# Autodesk Inventor assembly: trussstructure
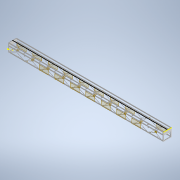
[picture p0: Inventor's stored thumbnail of the model, 180x180]
Saved by Autodesk Inventor 2020 (Build 240168000, 168)
## iProperties
Created: 2020-07-04
Part Number: trussstructure
Document SubType Name: Assembly
Designer: Ashiqrahman
Mass: 1909.65 g
Surface Area: 18631.2 cm^2
Volume: 1909.65 cm^3
Density: 1 g/cm^3
Author: Ashiqrahman
## Documents named in this file (12)
- D:\projects\Intelligent Picking\trussstructure.iam
- D:\projects\Intelligent Picking\LINK 2 tri truss without horizontal members.ipt
- C:\Users\Public\Documents\Autodesk\Inventor 2020\truss frame slanting.ipt
- C:\Users\Public\Documents\Autodesk\Inventor 2020\truss frame slanting down.ipt
- C:\Users\Public\Documents\Autodesk\Inventor 2020\truss final piece.ipt
- C:\Users\Public\Documents\Autodesk\Inventor 2020\horizontal bottom trusses.ipt
- C:\Users\Public\Documents\Autodesk\Inventor 2020\horizontal truss top.ipt
- D:\projects\Intelligent Picking\trussstructure\AIP\FEA\dajo7qeu8.fins
- D:\projects\Intelligent Picking\trussstructure\AIP\FEA\dajo7qeu8.fsat
- D:\projects\Intelligent Picking\trussstructure\AIP\FEA\dajo7qeu8.ftes
- D:\projects\Intelligent Picking\trussstructure\AIP\FEA\dajo7qeu8.fwiz
- D:\projects\Intelligent Picking\trussstructure\AIP\FEA\dajo7qeww.fmsh
## Components (60 placed, 6 different names)
1. LINK 2 tri truss without horizontal members:1 — Rotational:1, Mate:1, Mate:2, Mate:3, Flush:3, Flush:4, Mate:4, Mate:5, Flush:5, Mate:6, Mate:7, Mate:8, Mate:9, Flush:6, Mate:10, Mate:11, Flush:7, Mate:12, Mate:13, Flush:8, Mate:14, Mate:15, Flush:9, Mate:16, Mate:17, Flush:10, Mate:18, Mate:19, Flush:11, Mate:36, Mate:37, Flush:21, Mate:38, Mate:39, Flush:22, Mate:40, Flush:23, Mate:41, Mate:42, Flush:24, Mate:43, Mate:44, Mate:45, Mate:46, Mate:47, Flush:25, Mate:48, Mate:49, Flush:26, Mate:50, Mate:51, Flush:27, Mate:52, Mate:53, Flush:28, Mate:54, Mate:56, Mate:74, Flush:40, Mate:75, Flush:41, Mate:76, Mate:78, Flush:43, Flush:44, Flush:45, Mate:79, Mate:80, Flush:46, Mate:82, Mate:83, Flush:47, Mate:84, Mate:85, Flush:48, Mate:86, Mate:87, Mate:88, Flush:49, Mate:89, Mate:90, Flush:50, Mate:91, Mate:92, Flush:51, Mate:93, Mate:94, Flush:52, Mate:95, Mate:96, Flush:53, Mate:97, Mate:98, Flush:54, Flush:55, Flush:56, Mate:99, Mate:100, Flush:57, Mate:101, Mate:102, Flush:58, Mate:103, Mate:104, Flush:59, Mate:105, Mate:106, Flush:60, Mate:107, Mate:108, Flush:61, Mate:109, Mate:110, Flush:62, Mate:111, Mate:112, Flush:63, Mate:113, Mate:114, Flush:64, Mate:115, Mate:116, Flush:65
2. truss frame slanting:1 — Flush:2, Rotational:1, Mate:1, Mate:20
3. truss frame slanting down:1 — Flush:2, Mate:20, Mate:21
4. truss frame slanting:2 — Mate:2, Mate:3, Flush:3, Mate:21, Mate:22, Flush:12
5. truss frame slanting:3 — Mate:18, Mate:19, Flush:11, Mate:35, Mate:77, Flush:42
6. truss frame slanting:4 — Flush:4, Mate:4, Mate:5, Mate:23, Flush:13
7. truss frame slanting:5 — Mate:16, Mate:17, Flush:10, Mate:32, Mate:33, Flush:19
8. truss frame slanting:6 — Mate:12, Mate:13, Flush:8, Mate:28, Mate:29, Flush:17
9. truss frame slanting:7 — Mate:14, Mate:15, Flush:9, Mate:30, Mate:31, Flush:18
10. truss frame slanting:8 — Flush:5, Mate:6, Mate:7, Mate:24
11. truss frame slanting:9 — Mate:10, Mate:11, Flush:7, Mate:27, Flush:16
12. truss frame slanting:10 — Mate:8, Mate:9, Flush:6, Mate:25, Flush:14, Mate:26, Flush:15
13. truss frame slanting down:2 — Mate:24, Mate:25, Flush:14
14. truss frame slanting down:3 — Mate:23, Flush:13
15. truss frame slanting down:4 — Mate:22, Flush:12
16. truss frame slanting down:5 — Mate:26, Flush:15
17. truss frame slanting down:6 — Mate:27, Flush:16, Mate:28
18. truss frame slanting down:7 — Mate:29, Flush:17, Mate:30
19. truss frame slanting down:8 — Mate:31, Flush:18, Mate:32
20. truss frame slanting down:9 — Mate:33, Flush:19, Mate:35
21. truss frame slanting down:11 — Mate:44, Mate:45, Mate:46, Mate:64, Mate:65, Flush:34
22. truss frame slanting down:12 — Mate:40, Flush:23, Mate:41, Mate:60, Mate:61, Flush:32
23. truss frame slanting down:13 — Mate:36, Mate:37, Flush:21, Mate:55, Flush:29, Mate:58
24. truss frame slanting down:14 — Mate:38, Mate:39, Flush:22, Mate:57, Flush:30, Mate:59, Flush:31
25. truss frame slanting down:15 — Mate:42, Flush:24, Mate:43, Mate:62, Mate:63, Flush:33
26. truss frame slanting down:16 — Mate:47, Flush:25, Mate:48, Flush:35, Mate:66, Mate:67, Flush:36
27. truss frame slanting down:17 — Mate:49, Flush:26, Mate:50, Mate:68, Mate:69, Flush:37
28. truss frame slanting down:18 — Mate:51, Flush:27, Mate:52, Mate:70, Mate:71, Flush:38
29. truss frame slanting down:19 — Mate:53, Flush:28, Mate:54, Mate:72, Mate:73, Flush:39
30. truss frame slanting:11 — Mate:63, Flush:33, Mate:64
31. truss frame slanting:12 — Mate:65, Flush:34, Flush:35, Mate:66
32. truss frame slanting:13 — Mate:59, Flush:31, Mate:60
33. truss frame slanting:14 — Mate:55, Flush:29, Mate:56
34. truss frame slanting:15 — Mate:67, Flush:36, Mate:68
35. truss frame slanting:16 — Mate:61, Flush:32, Mate:62
36. truss frame slanting:17 — Mate:57, Flush:30, Mate:58
37. truss frame slanting:18 — Mate:69, Flush:37, Mate:70
38. truss frame slanting:19 — Mate:71, Flush:38, Mate:72
39. truss frame slanting:20 — Mate:73, Flush:39, Mate:74
40. truss final piece:1 — Flush:40, Mate:75, Flush:41, Mate:76
41. truss final piece:2 — Mate:77, Flush:42, Mate:78
42. horizontal bottom trusses:1 — Flush:43, Flush:44, Flush:45, Mate:79, Mate:80, Flush:46
43. horizontal bottom trusses:2 — Mate:91, Mate:92, Flush:51
44. horizontal bottom trusses:3 — Mate:84, Mate:85, Flush:48
45. horizontal bottom trusses:4 — Mate:89, Mate:90, Flush:50
46. horizontal bottom trusses:5 — Mate:86, Mate:87, Mate:88, Flush:49
47. horizontal bottom trusses:6 — Mate:95, Mate:96, Flush:53
48. horizontal bottom trusses:7 — Mate:93, Mate:94, Flush:52
49. horizontal bottom trusses:8 — Mate:82, Mate:83, Flush:47
50. horizontal bottom trusses:9 — Mate:97, Mate:98, Flush:54
51. horizontal truss top:1 — Flush:55, Flush:56
52. horizontal truss top:2 — Mate:99, Mate:100, Flush:57
53. horizontal truss top:3 — Mate:101, Mate:102, Flush:58
54. horizontal truss top:4 — Mate:103, Mate:104, Flush:59
55. horizontal truss top:5 — Mate:105, Mate:106, Flush:60
56. horizontal truss top:6 — Mate:107, Mate:108, Flush:61
57. horizontal truss top:7 — Mate:109, Mate:110, Flush:62
58. horizontal truss top:8 — Mate:111, Mate:112, Flush:63
59. horizontal truss top:9 — Mate:113, Mate:114, Flush:64
60. horizontal truss top:10 — Mate:115, Mate:116, Flush:65
## Relationships (178: Mate 114, Flush 63, RevoluteJoint 1)
- Flush:2: truss frame slanting:1 ↔ truss frame slanting down:1
- Rotational:1 [RevoluteJoint]: LINK 2 tri truss without horizontal members:1 ↔ truss frame slanting:1
- Mate:1: LINK 2 tri truss without horizontal members:1 ↔ truss frame slanting:1
- Mate:2: LINK 2 tri truss without horizontal members:1 ↔ truss frame slanting:2
- Mate:3: LINK 2 tri truss without horizontal members:1 ↔ truss frame slanting:2
- Flush:3 (-3 mm): LINK 2 tri truss without horizontal members:1 ↔ truss frame slanting:2
- Flush:4 (-3 mm): LINK 2 tri truss without horizontal members:1 ↔ truss frame slanting:4
- Mate:4: LINK 2 tri truss without horizontal members:1 ↔ truss frame slanting:4
- Mate:5: LINK 2 tri truss without horizontal members:1 ↔ truss frame slanting:4
- Flush:5 (-3 mm): LINK 2 tri truss without horizontal members:1 ↔ truss frame slanting:8
- Mate:6: LINK 2 tri truss without horizontal members:1 ↔ truss frame slanting:8
- Mate:7: LINK 2 tri truss without horizontal members:1 ↔ truss frame slanting:8
- Mate:8: LINK 2 tri truss without horizontal members:1 ↔ truss frame slanting:10
- Mate:9: LINK 2 tri truss without horizontal members:1 ↔ truss frame slanting:10
- Flush:6 (-3 mm): LINK 2 tri truss without horizontal members:1 ↔ truss frame slanting:10
- Mate:10: LINK 2 tri truss without horizontal members:1 ↔ truss frame slanting:9
- Mate:11: LINK 2 tri truss without horizontal members:1 ↔ truss frame slanting:9
- Flush:7 (-3 mm): LINK 2 tri truss without horizontal members:1 ↔ truss frame slanting:9
- Mate:12: LINK 2 tri truss without horizontal members:1 ↔ truss frame slanting:6
- Mate:13: LINK 2 tri truss without horizontal members:1 ↔ truss frame slanting:6
- Flush:8 (3 mm): LINK 2 tri truss without horizontal members:1 ↔ truss frame slanting:6
- Mate:14: LINK 2 tri truss without horizontal members:1 ↔ truss frame slanting:7
- Mate:15: LINK 2 tri truss without horizontal members:1 ↔ truss frame slanting:7
- Flush:9 (-3 mm): LINK 2 tri truss without horizontal members:1 ↔ truss frame slanting:7
- Mate:16: LINK 2 tri truss without horizontal members:1 ↔ truss frame slanting:5
- Mate:17: LINK 2 tri truss without horizontal members:1 ↔ truss frame slanting:5
- Flush:10 (-3 mm): LINK 2 tri truss without horizontal members:1 ↔ truss frame slanting:5
- Mate:18: LINK 2 tri truss without horizontal members:1 ↔ truss frame slanting:3
- Mate:19: LINK 2 tri truss without horizontal members:1 ↔ truss frame slanting:3
- Flush:11 (-3 mm): LINK 2 tri truss without horizontal members:1 ↔ truss frame slanting:3
- Mate:20: truss frame slanting:1 ↔ truss frame slanting down:1
- Mate:21: truss frame slanting down:1 ↔ truss frame slanting:2
- Mate:22: truss frame slanting:2 ↔ truss frame slanting down:4
- Flush:12 (3 mm): truss frame slanting:2 ↔ truss frame slanting down:4
- Mate:23: truss frame slanting:4 ↔ truss frame slanting down:3
- Flush:13 (-3 mm): truss frame slanting:4 ↔ truss frame slanting down:3
- Mate:24: truss frame slanting:8 ↔ truss frame slanting down:2
- Mate:25: truss frame slanting:10 ↔ truss frame slanting down:2
- Flush:14 (-3 mm): truss frame slanting:10 ↔ truss frame slanting down:2
- Mate:26: truss frame slanting:10 ↔ truss frame slanting down:5
- Flush:15 (-3 mm): truss frame slanting:10 ↔ truss frame slanting down:5
- Mate:27: truss frame slanting:9 ↔ truss frame slanting down:6
- Flush:16 (-3 mm): truss frame slanting:9 ↔ truss frame slanting down:6
- Mate:28: truss frame slanting:6 ↔ truss frame slanting down:6
- Mate:29: truss frame slanting:6 ↔ truss frame slanting down:7
- Flush:17 (-3 mm): truss frame slanting:6 ↔ truss frame slanting down:7
- Mate:30: truss frame slanting:7 ↔ truss frame slanting down:7
- Mate:31: truss frame slanting:7 ↔ truss frame slanting down:8
- Flush:18 (-3 mm): truss frame slanting:7 ↔ truss frame slanting down:8
- Mate:32: truss frame slanting:5 ↔ truss frame slanting down:8
- Mate:33: truss frame slanting:5 ↔ truss frame slanting down:9
- Flush:19 (3 mm): truss frame slanting:5 ↔ truss frame slanting down:9
- Mate:35: truss frame slanting:3 ↔ truss frame slanting down:9
- Mate:36: LINK 2 tri truss without horizontal members:1 ↔ truss frame slanting down:13
- Mate:37: LINK 2 tri truss without horizontal members:1 ↔ truss frame slanting down:13
- Flush:21 (-3 mm): LINK 2 tri truss without horizontal members:1 ↔ truss frame slanting down:13
- Mate:38: LINK 2 tri truss without horizontal members:1 ↔ truss frame slanting down:14
- Mate:39: LINK 2 tri truss without horizontal members:1 ↔ truss frame slanting down:14
- Flush:22 (-3 mm): LINK 2 tri truss without horizontal members:1 ↔ truss frame slanting down:14
- Mate:40: LINK 2 tri truss without horizontal members:1 ↔ truss frame slanting down:12
- Flush:23 (-3 mm): LINK 2 tri truss without horizontal members:1 ↔ truss frame slanting down:12
- Mate:41: LINK 2 tri truss without horizontal members:1 ↔ truss frame slanting down:12
- Mate:42: LINK 2 tri truss without horizontal members:1 ↔ truss frame slanting down:15
- Flush:24 (-3 mm): LINK 2 tri truss without horizontal members:1 ↔ truss frame slanting down:15
- Mate:43: LINK 2 tri truss without horizontal members:1 ↔ truss frame slanting down:15
- Mate:44: LINK 2 tri truss without horizontal members:1 ↔ truss frame slanting down:11
- Mate:45 (3 mm): LINK 2 tri truss without horizontal members:1 ↔ truss frame slanting down:11
- Mate:46: LINK 2 tri truss without horizontal members:1 ↔ truss frame slanting down:11
- Mate:47: LINK 2 tri truss without horizontal members:1 ↔ truss frame slanting down:16
- Flush:25 (-3 mm): LINK 2 tri truss without horizontal members:1 ↔ truss frame slanting down:16
- Mate:48: LINK 2 tri truss without horizontal members:1 ↔ truss frame slanting down:16
- Mate:49: LINK 2 tri truss without horizontal members:1 ↔ truss frame slanting down:17
- Flush:26 (-3 mm): LINK 2 tri truss without horizontal members:1 ↔ truss frame slanting down:17
- Mate:50: LINK 2 tri truss without horizontal members:1 ↔ truss frame slanting down:17
- Mate:51: LINK 2 tri truss without horizontal members:1 ↔ truss frame slanting down:18
- Flush:27 (-3 mm): LINK 2 tri truss without horizontal members:1 ↔ truss frame slanting down:18
- Mate:52: LINK 2 tri truss without horizontal members:1 ↔ truss frame slanting down:18
- Mate:53: LINK 2 tri truss without horizontal members:1 ↔ truss frame slanting down:19
- Flush:28 (-3 mm): LINK 2 tri truss without horizontal members:1 ↔ truss frame slanting down:19
- Mate:54: LINK 2 tri truss without horizontal members:1 ↔ truss frame slanting down:19
- Mate:55: truss frame slanting down:13 ↔ truss frame slanting:14
- Flush:29 (3 mm): truss frame slanting down:13 ↔ truss frame slanting:14
- Mate:56: LINK 2 tri truss without horizontal members:1 ↔ truss frame slanting:14
- Mate:57: truss frame slanting down:14 ↔ truss frame slanting:17
- Flush:30 (-3 mm): truss frame slanting down:14 ↔ truss frame slanting:17
- Mate:58: truss frame slanting down:13 ↔ truss frame slanting:17
- Mate:59: truss frame slanting down:14 ↔ truss frame slanting:13
- Flush:31 (-3 mm): truss frame slanting down:14 ↔ truss frame slanting:13
- Mate:60: truss frame slanting down:12 ↔ truss frame slanting:13
- Mate:61: truss frame slanting down:12 ↔ truss frame slanting:16
- Flush:32 (3 mm): truss frame slanting down:12 ↔ truss frame slanting:16
- Mate:62: truss frame slanting down:15 ↔ truss frame slanting:16
- Mate:63: truss frame slanting down:15 ↔ truss frame slanting:11
- Flush:33 (-3 mm): truss frame slanting down:15 ↔ truss frame slanting:11
- Mate:64: truss frame slanting down:11 ↔ truss frame slanting:11
- Mate:65: truss frame slanting down:11 ↔ truss frame slanting:12
- Flush:34 (3 mm): truss frame slanting down:11 ↔ truss frame slanting:12
- Flush:35 (-3 mm): truss frame slanting down:16 ↔ truss frame slanting:12
- Mate:66: truss frame slanting down:16 ↔ truss frame slanting:12
- Mate:67: truss frame slanting down:16 ↔ truss frame slanting:15
- Flush:36 (-3 mm): truss frame slanting down:16 ↔ truss frame slanting:15
- Mate:68: truss frame slanting down:17 ↔ truss frame slanting:15
- Mate:69: truss frame slanting down:17 ↔ truss frame slanting:18
- Flush:37 (3 mm): truss frame slanting down:17 ↔ truss frame slanting:18
- Mate:70: truss frame slanting down:18 ↔ truss frame slanting:18
- Mate:71: truss frame slanting down:18 ↔ truss frame slanting:19
- Flush:38 (3 mm): truss frame slanting down:18 ↔ truss frame slanting:19
- Mate:72: truss frame slanting down:19 ↔ truss frame slanting:19
- Mate:73: truss frame slanting down:19 ↔ truss frame slanting:20
- Flush:39 (3 mm): truss frame slanting down:19 ↔ truss frame slanting:20
- Mate:74: LINK 2 tri truss without horizontal members:1 ↔ truss frame slanting:20
- Flush:40: LINK 2 tri truss without horizontal members:1 ↔ truss final piece:1
- Mate:75: LINK 2 tri truss without horizontal members:1 ↔ truss final piece:1
- Flush:41 (-3 mm): LINK 2 tri truss without horizontal members:1 ↔ truss final piece:1
- Mate:76: LINK 2 tri truss without horizontal members:1 ↔ truss final piece:1
- Mate:77: truss frame slanting:3 ↔ truss final piece:2
- Flush:42 (-3 mm): truss frame slanting:3 ↔ truss final piece:2
- Mate:78: LINK 2 tri truss without horizontal members:1 ↔ truss final piece:2
- Flush:43: LINK 2 tri truss without horizontal members:1 ↔ horizontal bottom trusses:1
- Flush:44: LINK 2 tri truss without horizontal members:1 ↔ horizontal bottom trusses:1
- Flush:45: LINK 2 tri truss without horizontal members:1 ↔ horizontal bottom trusses:1
- Mate:79: LINK 2 tri truss without horizontal members:1 ↔ horizontal bottom trusses:1
- Mate:80: LINK 2 tri truss without horizontal members:1 ↔ horizontal bottom trusses:1
- Flush:46 (-3 mm): LINK 2 tri truss without horizontal members:1 ↔ horizontal bottom trusses:1
- Mate:82: LINK 2 tri truss without horizontal members:1 ↔ horizontal bottom trusses:8
- Mate:83: LINK 2 tri truss without horizontal members:1 ↔ horizontal bottom trusses:8
- Flush:47 (-3 mm): LINK 2 tri truss without horizontal members:1 ↔ horizontal bottom trusses:8
- Mate:84: LINK 2 tri truss without horizontal members:1 ↔ horizontal bottom trusses:3
- Mate:85: LINK 2 tri truss without horizontal members:1 ↔ horizontal bottom trusses:3
- Flush:48 (-3 mm): LINK 2 tri truss without horizontal members:1 ↔ horizontal bottom trusses:3
- Mate:86: LINK 2 tri truss without horizontal members:1 ↔ horizontal bottom trusses:5
- Mate:87: LINK 2 tri truss without horizontal members:1 ↔ horizontal bottom trusses:5
- Mate:88: LINK 2 tri truss without horizontal members:1 ↔ horizontal bottom trusses:5
- Flush:49 (-3 mm): LINK 2 tri truss without horizontal members:1 ↔ horizontal bottom trusses:5
- Mate:89: LINK 2 tri truss without horizontal members:1 ↔ horizontal bottom trusses:4
- Mate:90: LINK 2 tri truss without horizontal members:1 ↔ horizontal bottom trusses:4
- Flush:50 (-3 mm): LINK 2 tri truss without horizontal members:1 ↔ horizontal bottom trusses:4
- Mate:91: LINK 2 tri truss without horizontal members:1 ↔ horizontal bottom trusses:2
- Mate:92: LINK 2 tri truss without horizontal members:1 ↔ horizontal bottom trusses:2
- Flush:51 (-3 mm): LINK 2 tri truss without horizontal members:1 ↔ horizontal bottom trusses:2
- Mate:93: LINK 2 tri truss without horizontal members:1 ↔ horizontal bottom trusses:7
- Mate:94: LINK 2 tri truss without horizontal members:1 ↔ horizontal bottom trusses:7
- Flush:52 (-3 mm): LINK 2 tri truss without horizontal members:1 ↔ horizontal bottom trusses:7
- Mate:95: LINK 2 tri truss without horizontal members:1 ↔ horizontal bottom trusses:6
- Mate:96: LINK 2 tri truss without horizontal members:1 ↔ horizontal bottom trusses:6
- Flush:53 (-3 mm): LINK 2 tri truss without horizontal members:1 ↔ horizontal bottom trusses:6
- Mate:97: LINK 2 tri truss without horizontal members:1 ↔ horizontal bottom trusses:9
- Mate:98: LINK 2 tri truss without horizontal members:1 ↔ horizontal bottom trusses:9
- Flush:54 (-3 mm): LINK 2 tri truss without horizontal members:1 ↔ horizontal bottom trusses:9
- Flush:55: LINK 2 tri truss without horizontal members:1 ↔ horizontal truss top:1
- Flush:56: LINK 2 tri truss without horizontal members:1 ↔ horizontal truss top:1
- Mate:99: LINK 2 tri truss without horizontal members:1 ↔ horizontal truss top:2
- Mate:100: LINK 2 tri truss without horizontal members:1 ↔ horizontal truss top:2
- Flush:57 (-3 mm): LINK 2 tri truss without horizontal members:1 ↔ horizontal truss top:2
- Mate:101: LINK 2 tri truss without horizontal members:1 ↔ horizontal truss top:3
- Mate:102: LINK 2 tri truss without horizontal members:1 ↔ horizontal truss top:3
- Flush:58 (-3 mm): LINK 2 tri truss without horizontal members:1 ↔ horizontal truss top:3
- Mate:103: LINK 2 tri truss without horizontal members:1 ↔ horizontal truss top:4
- Mate:104: LINK 2 tri truss without horizontal members:1 ↔ horizontal truss top:4
- Flush:59 (-3 mm): LINK 2 tri truss without horizontal members:1 ↔ horizontal truss top:4
- Mate:105: LINK 2 tri truss without horizontal members:1 ↔ horizontal truss top:5
- Mate:106: LINK 2 tri truss without horizontal members:1 ↔ horizontal truss top:5
- Flush:60 (-3 mm): LINK 2 tri truss without horizontal members:1 ↔ horizontal truss top:5
- Mate:107: LINK 2 tri truss without horizontal members:1 ↔ horizontal truss top:6
- Mate:108: LINK 2 tri truss without horizontal members:1 ↔ horizontal truss top:6
- Flush:61 (-3 mm): LINK 2 tri truss without horizontal members:1 ↔ horizontal truss top:6
- Mate:109: LINK 2 tri truss without horizontal members:1 ↔ horizontal truss top:7
- Mate:110: LINK 2 tri truss without horizontal members:1 ↔ horizontal truss top:7
- Flush:62 (-3 mm): LINK 2 tri truss without horizontal members:1 ↔ horizontal truss top:7
- Mate:111: LINK 2 tri truss without horizontal members:1 ↔ horizontal truss top:8
- Mate:112: LINK 2 tri truss without horizontal members:1 ↔ horizontal truss top:8
- Flush:63 (-3 mm): LINK 2 tri truss without horizontal members:1 ↔ horizontal truss top:8
- Mate:113: LINK 2 tri truss without horizontal members:1 ↔ horizontal truss top:9
- Mate:114: LINK 2 tri truss without horizontal members:1 ↔ horizontal truss top:9
- Flush:64 (-3 mm): LINK 2 tri truss without horizontal members:1 ↔ horizontal truss top:9
- Mate:115: LINK 2 tri truss without horizontal members:1 ↔ horizontal truss top:10
- Mate:116: LINK 2 tri truss without horizontal members:1 ↔ horizontal truss top:10
- Flush:65 (3 mm): LINK 2 tri truss without horizontal members:1 ↔ horizontal truss top:10
## Named parameters: sa_0 = 10000, sa_1 = 981, sa_2 = 1000, sa_3 = 1000
note: some values were not read from the file. Shown as the stored number, unit unknown: "sa_0", "sa_1", "sa_2", "sa_3".
